# Autodesk Inventor assembly: R-wing
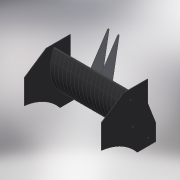
[picture p0: Inventor's stored thumbnail of the model, 180x180]
Saved by Autodesk Inventor 2018.2 (Build 222227000, 227)
## iProperties
Created: 2017-12-11
Part Number: R-wing
Material: 一般
Document SubType Name: Assembly
Designer: kuwano
Mass: 37579.8 g
Surface Area: 48667.5 cm^2
Volume: 32484 cm^3
Density: 1.15687 g/cm^3
Author: kuwano
## Documents named in this file (6)
- D:\kuwano\Documents\Inventor\KITformula\AeroCAD2018\CAD\Inventor\製作用CAD\R-wing\R-wing.iam
- D:\kuwano\Documents\Inventor\KITformula\AeroCAD2018\CAD\Inventor\製作用CAD\R-wing\parts\main_flap\main_flap.iam
- D:\kuwano\Documents\Inventor\KITformula\AeroCAD2018\CAD\Inventor\製作用CAD\R-wing\parts\end_plate.ipt
- D:\kuwano\Documents\Inventor\KITformula\AeroCAD2018\CAD\Inventor\製作用CAD\R-wing\parts\sub_flap\sub_flap.iam
- D:\kuwano\Documents\Inventor\KITformula\AeroCAD2018\CAD\Inventor\製作用CAD\R-wing\parts\swan_plate.ipt
- D:\kuwano\Documents\Inventor\KITformula\AeroCAD2018\CAD\Inventor\製作用CAD\R-wing\parts\joint\joint.iam
## Components (7 placed, 5 different names)
1. main_flap:1 [sub-assembly] — メイト:1, メイト:2, メイト:3, メイト:4, メイト:5, メイト:7, メイト:8, メイト:9, メイト:10, メイト:13, メイト:14, メイト:19
2. sub_flap:1 [sub-assembly] — メイト:11, メイト:12
3. end_plate:1 — メイト:1, フラッシュ:1, フラッシュ:2, メイト:9, メイト:10
4. end_plate:2 — メイト:2, フラッシュ:1, フラッシュ:2, メイト:7, メイト:8, メイト:11, メイト:12
5. swan_plate:1 — メイト:14, メイト:17, フラッシュ:3, フラッシュ:4, メイト:19, フラッシュ:5, メイト:20
6. swan_plate:2 — メイト:13, フラッシュ:3, フラッシュ:4, フラッシュ:5, フラッシュ:22
7. joint:1 [sub-assembly] — メイト:17, 角度:1, メイト:20, フラッシュ:22
## Relationships (23: Mate 16, Flush 6, Angle 1)
- メイト:1 [Mate]: main_flap:1 ↔ end_plate:1
- メイト:2 [Mate]: main_flap:1 ↔ end_plate:2
- フラッシュ:1 [Flush]: end_plate:1 ↔ end_plate:2
- フラッシュ:2 [Flush]: end_plate:1 ↔ end_plate:2
- メイト:3 [Mate]: main_flap:1
- メイト:4 [Mate]: main_flap:1
- メイト:5 [Mate]: main_flap:1
- メイト:7 [Mate]: main_flap:1 ↔ end_plate:2
- メイト:8 [Mate]: main_flap:1 ↔ end_plate:2
- メイト:9 [Mate]: main_flap:1 ↔ end_plate:1
- メイト:10 [Mate]: main_flap:1 ↔ end_plate:1
- メイト:11 [Mate]: sub_flap:1 ↔ end_plate:2
- メイト:12 [Mate]: sub_flap:1 ↔ end_plate:2
- メイト:13 [Mate]: main_flap:1 ↔ swan_plate:2
- メイト:14 [Mate]: main_flap:1 ↔ swan_plate:1
- メイト:17 [Mate]: swan_plate:1 ↔ joint:1
- フラッシュ:3 [Flush]: swan_plate:1 ↔ swan_plate:2
- フラッシュ:4 [Flush]: swan_plate:1 ↔ swan_plate:2
- メイト:19 [Mate]: main_flap:1 ↔ swan_plate:1
- フラッシュ:5 [Flush] (100 mm): swan_plate:1 ↔ swan_plate:2
- 角度:1 [Angle] (0 deg): joint:1
- メイト:20 [Mate]: swan_plate:1 ↔ joint:1
- フラッシュ:22 [Flush]: swan_plate:2 ↔ joint:1
